# Autodesk Inventor assembly: C10_ZP_top frame asm
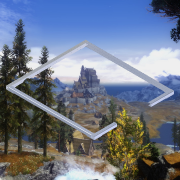
[picture p0: Inventor's stored thumbnail of the model, 180x180]
Saved by Autodesk Inventor 2015 SP1 (Build 190203100, 203)
## iProperties
Created: 2016-01-16
Part Number: C10_ZP_top frame asm
Document SubType Name: Assembly
Designer: Administrator
Mass: 1300.06 g
Surface Area: 4304.34 cm^2
Volume: 481.502 cm^3
Density: 2.7 g/cm^3
Author: Administrator
## Documents named in this file (5)
- G:\High School\First Robotics\2015-2016 Season\CAD\6-Wheel Big Sticky Chassis\C10_ZP_top frame asm.iam
- G:\High School\First Robotics\2015-2016 Season\CAD\6-Wheel Big Sticky Chassis\90 deg Gusset.ipt
- G:\High School\First Robotics\2015-2016 Season\CAD\6-Wheel Big Sticky Chassis\C6R1_ZP_side frame c-channel.ipt
- G:\High School\First Robotics\2015-2016 Season\CAD\6-Wheel Big Sticky Chassis\C8R1_ZP_front frames c-channel.ipt
- G:\High School\First Robotics\2015-2016 Season\CAD\6-Wheel Big Sticky Chassis\C7R1_ZP_back frame c-channel.ipt
## Components (9 placed, 4 different names)
1. C6R1_ZP_side frame c-channel:1 — Flush:2, Insert:1, Flush:7, Insert:8, Insert:11
2. C6R1_ZP_side frame c-channel:2 — Flush:3, Insert:2, Insert:4, Mate:9, Insert:10
3. C8R1_ZP_front frames c-channel:1 — Flush:3, Flush:8, Insert:13
4. C8R1_ZP_front frames c-channel:2 — Flush:2, Insert:3, Insert:12
5. 90 deg Gusset:1 — Insert:1, Insert:6, Insert:7, Insert:8
6. 90 deg Gusset:2 — Insert:3, Flush:7, Insert:11, Insert:12
7. 90 deg Gusset:3 — Insert:4, Flush:8, Insert:10, Insert:13
8. 90 deg Gusset:4 — Insert:2, Insert:5, Insert:9
9. C7R1_ZP_back frame c-channel:1 — Insert:5, Insert:6, Insert:7, Insert:9, Mate:9
## Relationships (18: Insert 13, Flush 4, Mate 1)
- Flush:2: C6R1_ZP_side frame c-channel:1 ↔ C8R1_ZP_front frames c-channel:2
- Flush:3: C6R1_ZP_side frame c-channel:2 ↔ C8R1_ZP_front frames c-channel:1
- Insert:1: C6R1_ZP_side frame c-channel:1 ↔ 90 deg Gusset:1
- Insert:2: C6R1_ZP_side frame c-channel:2 ↔ 90 deg Gusset:4
- Insert:3: C8R1_ZP_front frames c-channel:2 ↔ 90 deg Gusset:2
- Flush:7: C6R1_ZP_side frame c-channel:1 ↔ 90 deg Gusset:2
- Insert:4: C6R1_ZP_side frame c-channel:2 ↔ 90 deg Gusset:3
- Flush:8: C8R1_ZP_front frames c-channel:1 ↔ 90 deg Gusset:3
- Insert:5: 90 deg Gusset:4 ↔ C7R1_ZP_back frame c-channel:1
- Insert:6: 90 deg Gusset:1 ↔ C7R1_ZP_back frame c-channel:1
- Insert:7: 90 deg Gusset:1 ↔ C7R1_ZP_back frame c-channel:1
- Insert:8: C6R1_ZP_side frame c-channel:1 ↔ 90 deg Gusset:1
- Insert:9: 90 deg Gusset:4 ↔ C7R1_ZP_back frame c-channel:1
- Mate:9: C6R1_ZP_side frame c-channel:2 ↔ C7R1_ZP_back frame c-channel:1
- Insert:10: C6R1_ZP_side frame c-channel:2 ↔ 90 deg Gusset:3
- Insert:11: C6R1_ZP_side frame c-channel:1 ↔ 90 deg Gusset:2
- Insert:12: C8R1_ZP_front frames c-channel:2 ↔ 90 deg Gusset:2
- Insert:13: C8R1_ZP_front frames c-channel:1 ↔ 90 deg Gusset:3
